# Autodesk Inventor assembly: Alternate Z Drive Assembly
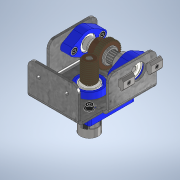
[picture p0: Inventor's stored thumbnail of the model, 180x180]
Saved by Autodesk Inventor 2022 (Build 260153000, 153)
## iProperties
Created: 2022-03-26
Part Number: Alternate Z Drive Assembly
Document SubType Name: Assembly
Designer: Nick
Author: Nick
## Documents named in this file (15)
- Y:\Projects\Bibble0\SubAsm\Alternate Z Drive Assembly.iam
- Y:\Projects\Bibble0\Bearings\625 Bearing.ipt
- Y:\Projects\Bibble0\3D printed\Motor to Bearing Adapter HSI.iam
- Y:\Projects\Bibble0\Sheet Metal\Z Drive Mount.ipt
- Y:\Projects\Bibble0\3D printed\Z Axis\Z Drive Bearing Holder.ipt
- Y:\Projects\Bibble0\Hardware\5 x 50mm Shaft.ipt
- Y:\Projects\Bibble0\Hardware\GT2 Pulley 16T.ipt
- Y:\Projects\Bibble0\Hardware\METAL WORM GEAR_57545K624 v5.ipt
- Y:\Projects\Bibble0\Hardware\PLASTIC WORM GEAR_4037N115 v3.ipt
- Y:\Projects\Bibble0\Hardware\M3 x 12 mm  SHCS.ipt
- Y:\Projects\Bibble0\Hardware\M3 T-Slot Nut.ipt
- Y:\Projects\Bibble0\Hardware\M3 x 6 mm SHCS.ipt
- Y:\Projects\Bibble0\Hardware\M3 Washer.ipt
- Y:\Projects\Bibble0\Hardware\5mm Collar.ipt
- Y:\Projects\Bibble0\Hardware\5mm to 8mm Coupler.iam
## Components (31 placed, 14 different names)
1. 625 Bearing:1 — Insert:1, Insert:30
2. 625 Bearing:2 — Insert:2
3. Motor to Bearing Adapter HSI:1 [sub-assembly] — Insert:1, Insert:2, Insert:28, Insert:29
4. Z Drive Mount:1 — Insert:28, Insert:29
5. Z Drive Bearing Holder:1
6. Z Drive Bearing Holder:2
7. 625 Bearing:3
8. 625 Bearing:4
9. 5 x 50mm Shaft:1
10. GT2 Pulley 16T:1
11. METAL WORM GEAR_57545K624 v5:1 — Insert:30, Insert:31
12. PLASTIC WORM GEAR_4037N115 v3:1
13. M3 x 12 mm  SHCS:1
14. M3 x 12 mm  SHCS:2
15. M3 x 12 mm  SHCS:3
16. M3 x 12 mm  SHCS:4
17. M3 T-Slot Nut:1
18. M3 T-Slot Nut:2
19. M3 T-Slot Nut:3
20. M3 T-Slot Nut:4
21. M3 x 6 mm SHCS:1
22. M3 Washer:1
23. M3 x 6 mm SHCS:2
24. M3 Washer:2
25. M3 x 6 mm SHCS:3
26. M3 Washer:3
27. M3 x 6 mm SHCS:4
28. M3 Washer:4
29. 5mm Collar:1
30. 5 x 50mm Shaft:2 — Insert:31, Insert:32
31. 5mm to 8mm Coupler:1 [sub-assembly] — Insert:32
## Relationships (40: Insert 29, Mate 6, Angle 4, Flush 1)
- Insert:1: 625 Bearing:1 ↔ Motor to Bearing Adapter HSI:1
- Insert:2: 625 Bearing:2 ↔ Motor to Bearing Adapter HSI:1
- [Insert]: Z Drive Bearing Holder:2 ↔ 625 Bearing:3
- [Insert]: Z Drive Bearing Holder:1 ↔ 625 Bearing:4
- [Mate]: 625 Bearing:4 ↔ 5 x 50mm Shaft:1
- [Flush]: 625 Bearing:4 ↔ 5 x 50mm Shaft:1
- [Insert]: GT2 Pulley 16T:1 ↔ PLASTIC WORM GEAR_4037N115 v3:1
- [Mate] (15 mm): Z Drive Bearing Holder:1 ↔ PLASTIC WORM GEAR_4037N115 v3:1
- [Mate]: 5 x 50mm Shaft:1 ↔ PLASTIC WORM GEAR_4037N115 v3:1
- [Mate]: 625 Bearing:3 ↔ 5 x 50mm Shaft:1
- [Insert]: Z Drive Mount:1 ↔ Z Drive Bearing Holder:1
- [Insert]: Z Drive Mount:1 ↔ Z Drive Bearing Holder:1
- [Insert]: Z Drive Mount:1 ↔ Z Drive Bearing Holder:2
- [Insert]: Z Drive Bearing Holder:2 ↔ M3 x 12 mm  SHCS:1
- [Insert]: Z Drive Bearing Holder:2 ↔ M3 x 12 mm  SHCS:3
- [Insert]: Z Drive Bearing Holder:1 ↔ M3 x 12 mm  SHCS:2
- [Insert]: Z Drive Bearing Holder:1 ↔ M3 x 12 mm  SHCS:4
- [Insert]: Z Drive Mount:1 ↔ M3 T-Slot Nut:4
- [Insert]: Z Drive Mount:1 ↔ M3 T-Slot Nut:1
- [Insert]: Z Drive Mount:1 ↔ M3 T-Slot Nut:3
- [Insert]: Z Drive Mount:1 ↔ M3 T-Slot Nut:2
- [Angle] (0 deg): M3 T-Slot Nut:2 ↔ M3 T-Slot Nut:3
- [Angle] (0 deg): Z Drive Mount:1 ↔ M3 T-Slot Nut:3
- [Angle] (0 deg): M3 T-Slot Nut:1 ↔ M3 T-Slot Nut:4
- [Angle] (0 deg): Z Drive Mount:1 ↔ M3 T-Slot Nut:1
- [Insert]: M3 x 6 mm SHCS:1 ↔ M3 Washer:1
- [Insert]: Z Drive Mount:1 ↔ M3 Washer:1
- [Insert]: M3 x 6 mm SHCS:2 ↔ M3 Washer:2
- [Insert]: M3 x 6 mm SHCS:3 ↔ M3 Washer:3
- [Insert]: M3 x 6 mm SHCS:4 ↔ M3 Washer:4
- [Insert]: Z Drive Mount:1 ↔ M3 Washer:2
- [Insert]: Z Drive Mount:1 ↔ M3 Washer:3
- [Insert]: Z Drive Mount:1 ↔ M3 Washer:4
- [Mate]: 625 Bearing:3 ↔ 5mm Collar:1
- [Mate]: 5 x 50mm Shaft:1 ↔ 5mm Collar:1
- Insert:28: Motor to Bearing Adapter HSI:1 ↔ Z Drive Mount:1
- Insert:29: Motor to Bearing Adapter HSI:1 ↔ Z Drive Mount:1
- Insert:30 (1 mm): 625 Bearing:1 ↔ METAL WORM GEAR_57545K624 v5:1
- Insert:31: METAL WORM GEAR_57545K624 v5:1 ↔ 5 x 50mm Shaft:2
- Insert:32: 5 x 50mm Shaft:2 ↔ 5mm to 8mm Coupler:1
## Named parameters: d33_d31 = 0 mm, d34_d31 = 0 mm, d35_d31 = 0 mm, d5_d36 = 0 mm, d6_d37 = 0 mm, d7_d38 = 0 mm, d10_d11 = 0 mm, d11_d12 = 0 mm, d12_d13 = 0 mm, d13_d14 = 0 mm, d18_d19 = 0 mm, d19_d20 = 0 mm, d20_d21 = 0 mm, d21_d22 = 0 mm, d22_d23 = 0 mm, d23_d24 = 0 mm, d24_d25 = 0 mm, d25_d26 = 0 mm, d26_d27 = 0 deg, d27_d28 = 0 deg, d28_d29 = 0 deg, d29_d30 = 0 deg, d30_d31 = 0 mm, d31_d32 = 0 mm
